# Autodesk Inventor assembly: vertical
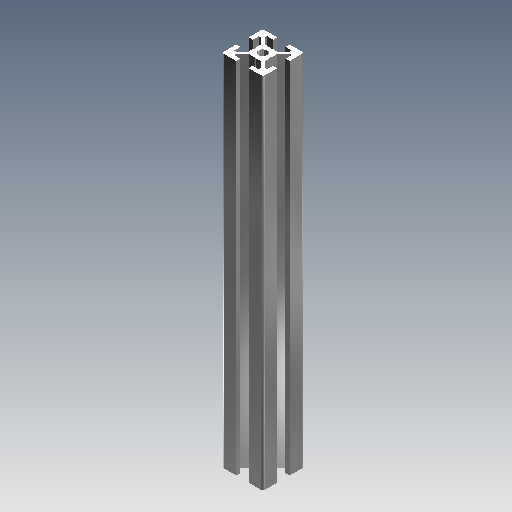
[picture p0: Inventor's stored thumbnail of the model, 512x512]
Saved by Autodesk Inventor 2017 (Build 210142000, 142)
## iProperties
Created: 2017-03-01
Part Number: vertical
Document SubType Name: Assembly
Designer: sawaiz
Author: sawaiz
## Documents named in this file (4)
- C:\Users\sawaiz\oneDrive\projects\sPhenixTileTestStand\frame\vertical.iam
- C:\Users\sawaiz\oneDrive\projects\sPhenixTileTestStand\frame\hfs5-2020Height.ipt
- C:\Users\sawaiz\oneDrive\projects\sPhenixTileTestStand\hardware\slideScrew.iam
- C:\Users\sawaiz\oneDrive\projects\sPhenixTileTestStand\sPhenixTileTestStand.xlsx
## Components (6 placed, 2 different names)
1. hfs5-2020Height:1 — Mate:1, Angle:1, Mate:2, Mate:3
2. slideScrew:1 [sub-assembly] — Mate:1, Angle:1, Mate:2, Mate:3
3. slideScrew:2 [sub-assembly]
4. slideScrew:3 [sub-assembly]
5. slideScrew:4 [sub-assembly]
6. slideScrew:5 [sub-assembly]
## Component patterns: (5 elements, first: slideScrew:1)
## Relationships (4: Mate 3, Angle 1)
- Mate:1: hfs5-2020Height:1 ↔ slideScrew:1
- Angle:1 (0 deg): hfs5-2020Height:1 ↔ slideScrew:1
- Mate:2 (1 mm): hfs5-2020Height:1 ↔ slideScrew:1
- Mate:3 (-17.5 mm): hfs5-2020Height:1 ↔ slideScrew:1
## Named parameters: plateWidth = 300 mm, plateDepth = 1000 mm, supportPlateThickness = 6.35 mm, supportPlateWidth = 50 mm, supportPlateFillet = 10 mm, separation = 35 mm, numPanels = 5, centerVerticalRatio = 0.3
